# Autodesk Inventor assembly: base_assembly
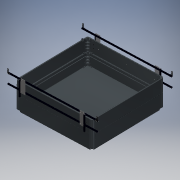
[picture p0: Inventor's stored thumbnail of the model, 180x180]
Saved by Autodesk Inventor 2018 (Build 220112000, 112)
## iProperties
Created: 2017-10-25
Part Number: base_assembly
Document SubType Name: Assembly
Designer: g
Author: g
## Documents named in this file (62)
- C:\Users\g\Desktop\AUG_inventor\base_assembly.iam
- C:\Users\g\Desktop\AUG_inventor\base_corner.ipt
- C:\Users\g\Desktop\AUG_inventor\base_wall.ipt
- C:\Users\g\Desktop\AUG_inventor\base_floor.ipt
- C:\Users\g\Desktop\AUG_inventor\makerbeam876mm.ipt
- C:\Users\g\Desktop\AUG_inventor\M3_Lock_Nut(Thin_Nut)_MIR.ipt
- C:\Users\g\Desktop\AUG_inventor\M3 X 10mm Screw_MIR.ipt
- C:\Users\g\Desktop\AUG_inventor\M3 X 10mm Screw_MIR2_MIR.ipt
- C:\Users\g\Desktop\AUG_inventor\M3_Lock_Nut(Thin_Nut)_MIR5_MIR.ipt
- C:\Users\g\Desktop\AUG_inventor\M3 X 20mm Screw_MIR_MIR_MIR1.ipt
- C:\Users\g\Desktop\AUG_inventor\M3_Lock_Nut(Thin_Nut)_MIR1_MIR_MIR1.ipt
- C:\Users\g\Desktop\AUG_inventor\makerbeam150mm_MIR_MIR_MIR_MIR1.ipt
- C:\Users\g\Desktop\AUG_inventor\M3 X 20mm Screw_MIR_MIR_MIR1_MIR.ipt
- C:\Users\g\Desktop\AUG_inventor\M3_Lock_Nut(Thin_Nut)_MIR1_MIR_MIR1_MIR.ipt
- C:\Users\g\Desktop\AUG_inventor\tieplate_small_MIR_MIR1.ipt
- C:\Users\g\Desktop\AUG_inventor\M3 X 10mm Screw_MIR2_MIR_MIR.ipt
- C:\Users\g\Desktop\AUG_inventor\M3_Lock_Nut(Thin_Nut)_MIR5_MIR_MIR.ipt
- C:\Users\g\Desktop\AUG_inventor\M3 X 20mm Screw_MIR_MIR_MIR1_MIR1.ipt
- C:\Users\g\Desktop\AUG_inventor\M3_Lock_Nut(Thin_Nut)_MIR1_MIR_MIR1_MIR1.ipt
- C:\Users\g\Desktop\AUG_inventor\makerbeam150mm_MIR_MIR_MIR_MIR1_MIR.ipt
- C:\Users\g\Desktop\AUG_inventor\M3 X 20mm Screw_MIR_MIR_MIR1_MIR_MIR.ipt
- C:\Users\g\Desktop\AUG_inventor\M3_Lock_Nut(Thin_Nut)_MIR1_MIR_MIR1_MIR_MIR.ipt
- C:\Users\g\Desktop\AUG_inventor\tieplate_small_MIR_MIR1_MIR.ipt
- C:\Users\g\Desktop\AUG_inventor\M3 X 10mm Screw_MIR2_MIR_MIR1.ipt
- C:\Users\g\Desktop\AUG_inventor\M3_Lock_Nut(Thin_Nut)_MIR5_MIR_MIR1.ipt
- C:\Users\g\Desktop\AUG_inventor\M3 X 10mm Screw_MIR2_MIR_MIR_MIR.ipt
- C:\Users\g\Desktop\AUG_inventor\M3_Lock_Nut(Thin_Nut)_MIR5_MIR_MIR_MIR.ipt
- C:\Users\g\Desktop\AUG_inventor\makerbeam876mm_MIR.ipt
- C:\Users\g\Desktop\AUG_inventor\M3_Lock_Nut(Thin_Nut)_MIR_MIR.ipt
- C:\Users\g\Desktop\AUG_inventor\M3 X 10mm Screw_MIR_MIR.ipt
- C:\Users\g\Desktop\AUG_inventor\M3 X 20mm Screw_MIR_MIR_MIR1_MIR2.ipt
- C:\Users\g\Desktop\AUG_inventor\M3_Lock_Nut(Thin_Nut)_MIR1_MIR_MIR1_MIR2.ipt
- C:\Users\g\Desktop\AUG_inventor\makerbeam150mm_MIR_MIR_MIR_MIR1_MIR1.ipt
- C:\Users\g\Desktop\AUG_inventor\M3 X 20mm Screw_MIR_MIR_MIR1_MIR_MIR1.ipt
- C:\Users\g\Desktop\AUG_inventor\M3_Lock_Nut(Thin_Nut)_MIR1_MIR_MIR1_MIR_MIR1.ipt
- C:\Users\g\Desktop\AUG_inventor\tieplate_small_MIR_MIR1_MIR1.ipt
- C:\Users\g\Desktop\AUG_inventor\M3 X 10mm Screw_MIR2_MIR_MIR2.ipt
- C:\Users\g\Desktop\AUG_inventor\M3_Lock_Nut(Thin_Nut)_MIR5_MIR_MIR2.ipt
- C:\Users\g\Desktop\AUG_inventor\M3 X 10mm Screw_MIR2_MIR_MIR_MIR1.ipt
- C:\Users\g\Desktop\AUG_inventor\M3_Lock_Nut(Thin_Nut)_MIR5_MIR_MIR_MIR1.ipt
- C:\Users\g\Desktop\AUG_inventor\M3 X 20mm Screw_MIR_MIR_MIR1_MIR1_MIR.ipt
- C:\Users\g\Desktop\AUG_inventor\M3_Lock_Nut(Thin_Nut)_MIR1_MIR_MIR1_MIR1_MIR.ipt
- C:\Users\g\Desktop\AUG_inventor\makerbeam150mm_MIR_MIR_MIR_MIR1_MIR_MIR.ipt
- C:\Users\g\Desktop\AUG_inventor\M3 X 20mm Screw_MIR_MIR_MIR1_MIR_MIR_MIR.ipt
- C:\Users\g\Desktop\AUG_inventor\M3_Lock_Nut(Thin_Nut)_MIR1_MIR_MIR1_MIR_MIR_MIR.ipt
- C:\Users\g\Desktop\AUG_inventor\tieplate_small_MIR_MIR1_MIR_MIR.ipt
- C:\Users\g\Desktop\AUG_inventor\M3 X 10mm Screw_MIR2_MIR_MIR1_MIR.ipt
- C:\Users\g\Desktop\AUG_inventor\M3_Lock_Nut(Thin_Nut)_MIR5_MIR_MIR1_MIR.ipt
- C:\Users\g\Desktop\AUG_inventor\M3 X 10mm Screw_MIR2_MIR_MIR_MIR_MIR.ipt
- C:\Users\g\Desktop\AUG_inventor\M3_Lock_Nut(Thin_Nut)_MIR5_MIR_MIR_MIR_MIR.ipt
- C:\Users\g\Desktop\AUG_inventor\makerbeam_L-bracket.ipt
- C:\Users\g\Desktop\AUG_inventor\M3_Lock_Nut(Thin_Nut).ipt
- C:\Users\g\Desktop\AUG_inventor\M3 X 10mm Screw.ipt
- C:\Users\g\Desktop\AUG_inventor\makerbeam_L-bracket_MIR2.ipt
- C:\Users\g\Desktop\AUG_inventor\M3_Lock_Nut(Thin_Nut)_MIR6.ipt
- C:\Users\g\Desktop\AUG_inventor\M3 X 10mm Screw_MIR3.ipt
- C:\Users\g\Desktop\AUG_inventor\makerbeam_L-bracket_MIR3.ipt
- C:\Users\g\Desktop\AUG_inventor\M3_Lock_Nut(Thin_Nut)_MIR7.ipt
- C:\Users\g\Desktop\AUG_inventor\M3 X 10mm Screw_MIR4.ipt
- C:\Users\g\Desktop\AUG_inventor\makerbeam_L-bracket_MIR2_MIR.ipt
- C:\Users\g\Desktop\AUG_inventor\M3_Lock_Nut(Thin_Nut)_MIR6_MIR.ipt
- C:\Users\g\Desktop\AUG_inventor\M3 X 10mm Screw_MIR3_MIR.ipt
## Components (117 placed, 61 different names)
1. base_wall:2 — Mate:1, Mate:2, Mate:9, Mate:10, Mate:15, Mate:16, Mate:23, Mate:61, Mate:62, Mate:67, Mate:68, Mate:69, Mate:114, Mate:170
2. base_wall:3 — Mate:11, Mate:12, Mate:13, Mate:14, Mate:22, Mate:57, Mate:58, Mate:63, Mate:64, Mate:70, Mate:113, Mate:123, Mate:124, Flush:2, Mate:133, Mate:145, Mate:149, Mate:164, Mate:168
3. base_wall:4 — Mate:3, Mate:4, Mate:5, Mate:6, Mate:17, Mate:18, Mate:19, Mate:24, Mate:25, Mate:60, Mate:65, Mate:66, Mate:134, Mate:135
4. base_corner:4 — Mate:1, Mate:2, Mate:3, Mate:4, Mate:16, Mate:17, Mate:23, Mate:60, Mate:61, Mate:66, Mate:67
5. base_corner:5 — Mate:13, Mate:14, Mate:57, Mate:58, Mate:64
6. base_corner:6 — Mate:5, Mate:6, Mate:7, Mate:8, Mate:18, Mate:19, Mate:20, Mate:21, Mate:24, Mate:25, Mate:26, Mate:27, Mate:28, Mate:59, Mate:65
7. base_corner:7 — Mate:9, Mate:10, Mate:11, Mate:12, Mate:15, Mate:22, Mate:62, Mate:63, Mate:68, Mate:69, Mate:70, Flush:1
8. base_wall:5 — Mate:7, Mate:8, Mate:20, Mate:21, Mate:26, Mate:27, Mate:28, Mate:59, Mate:169
9. base_wall:6 — Mate:114, Mate:116, Mate:121
10. base_wall:7 — Mate:113, Mate:118
11. base_wall:8 — Mate:122
12. base_corner:8
13. base_corner:9
14. base_corner:10
15. base_corner:11
16. base_wall:9 — Mate:117, Mate:171
17. base_floor:1 — Mate:121, Mate:122
18. makerbeam876mm:1 — Mate:124, Flush:1, Flush:2, Rigid:1, Flush:27, Mate:165, Mate:166, Mate:167, Slider:21, Flush:32, Symmetry:2
19. makerbeam876mm:4 — Rigid:1, Flush:27, Flush:28, Mate:162, Flush:29, Slider:22, Slider:23, Flush:33, Mate:173, Symmetry:2
20. M3_Lock_Nut(Thin_Nut)_MIR:1 — Slider:21, Flush:32, Cylindrical:20
21. M3_Lock_Nut(Thin_Nut)_MIR:2 — Rotational:3
22. M3_Lock_Nut(Thin_Nut)_MIR:3 — Rigid:4
23. M3 X 10mm Screw_MIR:1 — Rotational:3, Mate:145
24. M3 X 10mm Screw_MIR:2 — Cylindrical:20, Mate:168
25. M3 X 10mm Screw_MIR:3 — Rigid:4, Mate:149
26. M3 X 20mm Screw_MIR_MIR_MIR1:1 — Cylindrical:18, Mate:164
27. M3_Lock_Nut(Thin_Nut)_MIR1_MIR_MIR1:1 — Slider:20, Flush:31, Cylindrical:18
28. makerbeam150mm_MIR_MIR_MIR_MIR1:1 — Flush:28, Mate:162, Flush:29, Slider:20, Flush:31, Mate:172, Mate:174
29. M3 X 20mm Screw_MIR_MIR_MIR1_MIR:1 — Cylindrical:19
30. M3_Lock_Nut(Thin_Nut)_MIR1_MIR_MIR1_MIR:1 — Cylindrical:19
31. tieplate_small_MIR_MIR1:1 — Flush:33, Mate:173, Mate:174, Mate:175, Mate:176, Mate:177
32. M3 X 10mm Screw_MIR2_MIR:1 — Cylindrical:22, Mate:176
33. M3_Lock_Nut(Thin_Nut)_MIR5_MIR:1 — Slider:23, Cylindrical:22, Mate:175
34. M3_Lock_Nut(Thin_Nut)_MIR5_MIR:2 — Slider:22, Mate:172, Cylindrical:21
35. M3 X 10mm Screw_MIR2_MIR:2 — Cylindrical:21, Mate:177
36. M3 X 10mm Screw_MIR2_MIR_MIR:1 — Cylindrical:23
37. M3_Lock_Nut(Thin_Nut)_MIR5_MIR_MIR:1 — Cylindrical:23
38. M3_Lock_Nut(Thin_Nut)_MIR5_MIR_MIR:2 — Cylindrical:24
39. M3 X 10mm Screw_MIR2_MIR_MIR:2 — Cylindrical:24
40. M3 X 20mm Screw_MIR_MIR_MIR1_MIR1:1 — Cylindrical:25
41. M3_Lock_Nut(Thin_Nut)_MIR1_MIR_MIR1_MIR1:1 — Flush:34, Cylindrical:25, Slider:24
42. makerbeam150mm_MIR_MIR_MIR_MIR1_MIR:1 — Flush:34, Mate:178, Mate:181, Slider:24
43. M3 X 20mm Screw_MIR_MIR_MIR1_MIR_MIR:1 — Cylindrical:26
44. M3_Lock_Nut(Thin_Nut)_MIR1_MIR_MIR1_MIR_MIR:1 — Cylindrical:26
45. tieplate_small_MIR_MIR1_MIR:1 — Mate:178, Mate:179, Mate:180, Mate:182
46. M3 X 10mm Screw_MIR2_MIR_MIR1:1 — Mate:179, Cylindrical:27
47. M3_Lock_Nut(Thin_Nut)_MIR5_MIR_MIR1:1 — Mate:180, Cylindrical:27
48. M3_Lock_Nut(Thin_Nut)_MIR5_MIR_MIR1:2 — Mate:181, Cylindrical:28
49. M3 X 10mm Screw_MIR2_MIR_MIR1:2 — Mate:182, Cylindrical:28
50. M3 X 10mm Screw_MIR2_MIR_MIR_MIR:1 — Cylindrical:29
51. M3_Lock_Nut(Thin_Nut)_MIR5_MIR_MIR_MIR:1 — Cylindrical:29
52. M3_Lock_Nut(Thin_Nut)_MIR5_MIR_MIR_MIR:2 — Cylindrical:30
53. M3 X 10mm Screw_MIR2_MIR_MIR_MIR:2 — Cylindrical:30
54. makerbeam876mm_MIR:1 — Flush:35, Flush:36, Mate:184, Mate:185, Mate:186, Symmetry:3, Rigid:5, Slider:25
55. makerbeam876mm_MIR:2 — Flush:35, Flush:38, Mate:183, Flush:39, Mate:188, Flush:40, Symmetry:3, Rigid:5, Slider:27, Slider:28, Slider:30, Flush:42, Slider:31, Mate:198, Flush:43, Flush:44
56. M3_Lock_Nut(Thin_Nut)_MIR_MIR:1 — Flush:36, Slider:25, Cylindrical:31
57. M3_Lock_Nut(Thin_Nut)_MIR_MIR:2 — Rotational:4
58. M3_Lock_Nut(Thin_Nut)_MIR_MIR:3 — Rigid:6
59. M3 X 10mm Screw_MIR_MIR:1 — Rotational:4
60. M3 X 10mm Screw_MIR_MIR:2 — Cylindrical:31
61. M3 X 10mm Screw_MIR_MIR:3 — Rigid:6
62. M3 X 20mm Screw_MIR_MIR_MIR1_MIR2:1 — Cylindrical:32
63. M3_Lock_Nut(Thin_Nut)_MIR1_MIR_MIR1_MIR2:1 — Flush:37, Cylindrical:32, Slider:26
64. makerbeam150mm_MIR_MIR_MIR_MIR1_MIR1:1 — Flush:37, Flush:38, Mate:183, Flush:39, Mate:187, Mate:191, Slider:26
65. M3 X 20mm Screw_MIR_MIR_MIR1_MIR_MIR1:1 — Cylindrical:33
66. M3_Lock_Nut(Thin_Nut)_MIR1_MIR_MIR1_MIR_MIR1:1 — Cylindrical:33
67. tieplate_small_MIR_MIR1_MIR1:1 — Mate:187, Mate:188, Flush:40, Mate:189, Mate:190, Mate:192
68. M3 X 10mm Screw_MIR2_MIR_MIR2:1 — Mate:189, Cylindrical:34
69. M3_Lock_Nut(Thin_Nut)_MIR5_MIR_MIR2:1 — Mate:190, Cylindrical:34, Slider:27
70. M3_Lock_Nut(Thin_Nut)_MIR5_MIR_MIR2:2 — Mate:191, Slider:28, Cylindrical:35
71. M3 X 10mm Screw_MIR2_MIR_MIR2:2 — Mate:192, Cylindrical:35
72. M3 X 10mm Screw_MIR2_MIR_MIR_MIR1:1 — Cylindrical:36
73. M3_Lock_Nut(Thin_Nut)_MIR5_MIR_MIR_MIR1:1 — Cylindrical:36
74. M3_Lock_Nut(Thin_Nut)_MIR5_MIR_MIR_MIR1:2 — Cylindrical:37
75. M3 X 10mm Screw_MIR2_MIR_MIR_MIR1:2 — Cylindrical:37
76. M3 X 20mm Screw_MIR_MIR_MIR1_MIR1_MIR:1 — Cylindrical:38
77. M3_Lock_Nut(Thin_Nut)_MIR1_MIR_MIR1_MIR1_MIR:1 — Flush:41, Cylindrical:38, Slider:29
78. makerbeam150mm_MIR_MIR_MIR_MIR1_MIR_MIR:1 — Flush:41, Mate:193, Mate:196, Slider:29
79. M3 X 20mm Screw_MIR_MIR_MIR1_MIR_MIR_MIR:1 — Cylindrical:39
80. M3_Lock_Nut(Thin_Nut)_MIR1_MIR_MIR1_MIR_MIR_MIR:1 — Cylindrical:39
81. tieplate_small_MIR_MIR1_MIR_MIR:1 — Mate:193, Mate:194, Mate:195, Mate:197
82. M3 X 10mm Screw_MIR2_MIR_MIR1_MIR:1 — Mate:194, Cylindrical:40
83. M3_Lock_Nut(Thin_Nut)_MIR5_MIR_MIR1_MIR:1 — Mate:195, Cylindrical:40
84. M3_Lock_Nut(Thin_Nut)_MIR5_MIR_MIR1_MIR:2 — Mate:196, Cylindrical:41
85. M3 X 10mm Screw_MIR2_MIR_MIR1_MIR:2 — Mate:197, Cylindrical:41
86. M3 X 10mm Screw_MIR2_MIR_MIR_MIR_MIR:1 — Cylindrical:42
87. M3_Lock_Nut(Thin_Nut)_MIR5_MIR_MIR_MIR_MIR:1 — Cylindrical:42
88. M3_Lock_Nut(Thin_Nut)_MIR5_MIR_MIR_MIR_MIR:2 — Cylindrical:43
89. M3 X 10mm Screw_MIR2_MIR_MIR_MIR_MIR:2 — Cylindrical:43
90. makerbeam_L-bracket:1 — Mate:198, Flush:43, Flush:44, Mate:199, Mate:200, Mate:201, Mate:202, Cylindrical:46, Mate:203
91. M3_Lock_Nut(Thin_Nut):1 — Slider:30, Flush:42, Cylindrical:45
92. M3_Lock_Nut(Thin_Nut):2 — Slider:31, Mate:199, Cylindrical:44
93. M3 X 10mm Screw:1 — Cylindrical:44, Mate:200
94. M3 X 10mm Screw:2 — Cylindrical:45, Mate:201
95. M3_Lock_Nut(Thin_Nut):3 — Mate:202
96. M3 X 10mm Screw:3 — Cylindrical:46, Mate:203
97. makerbeam_L-bracket_MIR2:1 — Mate:204, Mate:205, Mate:206, Mate:207, Mate:208, Cylindrical:49
98. M3_Lock_Nut(Thin_Nut)_MIR6:1 — Cylindrical:48
99. M3_Lock_Nut(Thin_Nut)_MIR6:2 — Mate:204, Cylindrical:47
100. M3 X 10mm Screw_MIR3:1 — Mate:205, Cylindrical:47
101. M3 X 10mm Screw_MIR3:2 — Mate:206, Cylindrical:48
102. M3_Lock_Nut(Thin_Nut)_MIR6:3 — Mate:207
103. M3 X 10mm Screw_MIR3:3 — Mate:208, Cylindrical:49
104. makerbeam_L-bracket_MIR3:1 — Mate:209, Mate:210, Mate:211, Mate:212, Mate:213, Cylindrical:52
105. M3_Lock_Nut(Thin_Nut)_MIR7:1 — Cylindrical:51
106. M3_Lock_Nut(Thin_Nut)_MIR7:2 — Mate:209, Cylindrical:50
107. M3 X 10mm Screw_MIR4:1 — Mate:210, Cylindrical:50
108. M3 X 10mm Screw_MIR4:2 — Mate:211, Cylindrical:51
109. M3_Lock_Nut(Thin_Nut)_MIR7:3 — Mate:212
110. M3 X 10mm Screw_MIR4:3 — Mate:213, Cylindrical:52
111. makerbeam_L-bracket_MIR2_MIR:1 — Mate:214, Mate:215, Mate:216, Mate:217, Mate:218, Cylindrical:55
112. M3_Lock_Nut(Thin_Nut)_MIR6_MIR:1 — Cylindrical:54
113. M3_Lock_Nut(Thin_Nut)_MIR6_MIR:2 — Mate:214, Cylindrical:53
114. M3 X 10mm Screw_MIR3_MIR:1 — Mate:215, Cylindrical:53
115. M3 X 10mm Screw_MIR3_MIR:2 — Mate:216, Cylindrical:54
116. M3_Lock_Nut(Thin_Nut)_MIR6_MIR:3 — Mate:217
117. M3 X 10mm Screw_MIR3_MIR:3 — Mate:218, Cylindrical:55
## Relationships (233: Mate 156, CylindricalJoint 38, Flush 19, TranslationJoint 12, WeldJoint 4, RevoluteJoint 2, Symmetry 2)
- Mate:1: base_wall:2 ↔ base_corner:4
- Mate:2: base_wall:2 ↔ base_corner:4
- Mate:3: base_wall:4 ↔ base_corner:4
- Mate:4: base_wall:4 ↔ base_corner:4
- Mate:5: base_wall:4 ↔ base_corner:6
- Mate:6: base_wall:4 ↔ base_corner:6
- Mate:7: base_corner:6 ↔ base_wall:5
- Mate:8: base_corner:6 ↔ base_wall:5
- Mate:9: base_wall:2 ↔ base_corner:7
- Mate:10: base_wall:2 ↔ base_corner:7
- Mate:11: base_wall:3 ↔ base_corner:7
- Mate:12: base_wall:3 ↔ base_corner:7
- Mate:13: base_wall:3 ↔ base_corner:5
- Mate:14: base_wall:3 ↔ base_corner:5
- Mate:15: base_wall:2 ↔ base_corner:7
- Mate:16: base_wall:2 ↔ base_corner:4
- Mate:17: base_wall:4 ↔ base_corner:4
- Mate:18: base_wall:4 ↔ base_corner:6
- Mate:19: base_wall:4 ↔ base_corner:6
- Mate:20: base_corner:6 ↔ base_wall:5
- Mate:21: base_corner:6 ↔ base_wall:5
- Mate:22: base_wall:3 ↔ base_corner:7
- Mate:23: base_wall:2 ↔ base_corner:4
- Mate:24: base_wall:4 ↔ base_corner:6
- Mate:25: base_wall:4 ↔ base_corner:6
- Mate:26: base_corner:6 ↔ base_wall:5
- Mate:27: base_corner:6 ↔ base_wall:5
- Mate:28: base_corner:6 ↔ base_wall:5
- Mate:57: base_wall:3 ↔ base_corner:5
- Mate:58: base_wall:3 ↔ base_corner:5
- Mate:59: base_corner:6 ↔ base_wall:5
- Mate:60: base_wall:4 ↔ base_corner:4
- Mate:61: base_wall:2 ↔ base_corner:4
- Mate:62: base_wall:2 ↔ base_corner:7
- Mate:63: base_wall:3 ↔ base_corner:7
- Mate:64: base_wall:3 ↔ base_corner:5
- Mate:65: base_wall:4 ↔ base_corner:6
- Mate:66: base_wall:4 ↔ base_corner:4
- Mate:67: base_wall:2 ↔ base_corner:4
- Mate:68: base_wall:2 ↔ base_corner:7
- Mate:69: base_wall:2 ↔ base_corner:7
- Mate:70: base_wall:3 ↔ base_corner:7
- [Mate]: base_wall:6 ↔ base_corner:8
- [Mate]: base_wall:6 ↔ base_corner:8
- [Mate]: base_wall:8 ↔ base_corner:8
- [Mate]: base_wall:8 ↔ base_corner:8
- [Mate]: base_wall:8 ↔ base_corner:10
- [Mate]: base_wall:8 ↔ base_corner:10
- [Mate]: base_corner:10 ↔ base_wall:9
- [Mate]: base_corner:10 ↔ base_wall:9
- [Mate]: base_wall:6 ↔ base_corner:11
- [Mate]: base_wall:6 ↔ base_corner:11
- [Mate]: base_wall:7 ↔ base_corner:11
- [Mate]: base_wall:7 ↔ base_corner:11
- [Mate]: base_wall:7 ↔ base_corner:9
- [Mate]: base_wall:7 ↔ base_corner:9
- [Mate]: base_wall:6 ↔ base_corner:11
- [Mate]: base_wall:6 ↔ base_corner:8
- [Mate]: base_wall:8 ↔ base_corner:8
- [Mate]: base_wall:8 ↔ base_corner:10
- [Mate]: base_wall:8 ↔ base_corner:10
- [Mate]: base_corner:10 ↔ base_wall:9
- [Mate]: base_corner:10 ↔ base_wall:9
- [Mate]: base_wall:7 ↔ base_corner:11
- [Mate]: base_wall:6 ↔ base_corner:8
- [Mate]: base_wall:8 ↔ base_corner:10
- [Mate]: base_wall:8 ↔ base_corner:10
- [Mate]: base_corner:10 ↔ base_wall:9
- [Mate]: base_corner:10 ↔ base_wall:9
- [Mate]: base_corner:10 ↔ base_wall:9
- [Mate]: base_wall:7 ↔ base_corner:9
- [Mate]: base_wall:7 ↔ base_corner:9
- [Mate]: base_corner:10 ↔ base_wall:9
- [Mate]: base_wall:8 ↔ base_corner:8
- [Mate]: base_wall:6 ↔ base_corner:8
- [Mate]: base_wall:6 ↔ base_corner:11
- [Mate]: base_wall:7 ↔ base_corner:11
- [Mate]: base_wall:7 ↔ base_corner:9
- [Mate]: base_wall:8 ↔ base_corner:10
- [Mate]: base_wall:8 ↔ base_corner:8
- [Mate]: base_wall:6 ↔ base_corner:8
- [Mate]: base_wall:6 ↔ base_corner:11
- [Mate]: base_wall:6 ↔ base_corner:11
- [Mate]: base_wall:7 ↔ base_corner:11
- Mate:113: base_wall:3 ↔ base_wall:7
- Mate:114: base_wall:2 ↔ base_wall:6
- Mate:116: base_wall:6
- Mate:117: base_wall:9
- Mate:118: base_wall:7
- Mate:119
- Mate:120
- Mate:121: base_wall:6 ↔ base_floor:1
- Mate:122: base_wall:8 ↔ base_floor:1
- Mate:123: base_wall:3
- Mate:124 (5 mm): base_wall:3 ↔ makerbeam876mm:1
- Flush:1 (-68 mm): base_corner:7 ↔ makerbeam876mm:1
- Flush:2 (57.5 mm): base_wall:3 ↔ makerbeam876mm:1
- Rigid:1 [WeldJoint] (85 mm): makerbeam876mm:1 ↔ makerbeam876mm:4
- Rotational:3 [RevoluteJoint] (2.55 mm): M3_Lock_Nut(Thin_Nut)_MIR:2 ↔ M3 X 10mm Screw_MIR:1
- Rigid:4 [WeldJoint] (-2.54 mm): M3_Lock_Nut(Thin_Nut)_MIR:3 ↔ M3 X 10mm Screw_MIR:3
- Mate:133: base_wall:3
- Mate:134: base_wall:4
- Mate:135: base_wall:4
- Mate:145: base_wall:3 ↔ M3 X 10mm Screw_MIR:1
- Mate:149: base_wall:3 ↔ M3 X 10mm Screw_MIR:3
- Flush:27: makerbeam876mm:1 ↔ makerbeam876mm:4
- Flush:28: makerbeam876mm:4 ↔ makerbeam150mm_MIR_MIR_MIR_MIR1:1
- Mate:162: makerbeam876mm:4 ↔ makerbeam150mm_MIR_MIR_MIR_MIR1:1
- Flush:29 (120 mm): makerbeam876mm:4 ↔ makerbeam150mm_MIR_MIR_MIR_MIR1:1
- Slider:20 [TranslationJoint] (0.25 mm): M3_Lock_Nut(Thin_Nut)_MIR1_MIR_MIR1:1 ↔ makerbeam150mm_MIR_MIR_MIR_MIR1:1
- Flush:31 (80 mm): M3_Lock_Nut(Thin_Nut)_MIR1_MIR_MIR1:1 ↔ makerbeam150mm_MIR_MIR_MIR_MIR1:1
- Cylindrical:18: M3 X 20mm Screw_MIR_MIR_MIR1:1 ↔ M3_Lock_Nut(Thin_Nut)_MIR1_MIR_MIR1:1
- Mate:164: base_wall:3 ↔ M3 X 20mm Screw_MIR_MIR_MIR1:1
- Mate:165: makerbeam876mm:1
- Mate:166: makerbeam876mm:1
- Mate:167: makerbeam876mm:1
- Cylindrical:19: M3 X 20mm Screw_MIR_MIR_MIR1_MIR:1 ↔ M3_Lock_Nut(Thin_Nut)_MIR1_MIR_MIR1_MIR:1
- Slider:21 [TranslationJoint]: makerbeam876mm:1 ↔ M3_Lock_Nut(Thin_Nut)_MIR:1
- Flush:32 (168 mm): makerbeam876mm:1 ↔ M3_Lock_Nut(Thin_Nut)_MIR:1
- Cylindrical:20: M3_Lock_Nut(Thin_Nut)_MIR:1 ↔ M3 X 10mm Screw_MIR:2
- Mate:168: base_wall:3 ↔ M3 X 10mm Screw_MIR:2
- Mate:169: base_wall:5
- Mate:170: base_wall:2
- Mate:171: base_wall:9
- Slider:22 [TranslationJoint]: makerbeam876mm:4 ↔ M3_Lock_Nut(Thin_Nut)_MIR5_MIR:2
- Mate:172 (5 mm): makerbeam150mm_MIR_MIR_MIR_MIR1:1 ↔ M3_Lock_Nut(Thin_Nut)_MIR5_MIR:2
- Slider:23 [TranslationJoint]: makerbeam876mm:4 ↔ M3_Lock_Nut(Thin_Nut)_MIR5_MIR:1
- Flush:33 (-10 mm): makerbeam876mm:4 ↔ tieplate_small_MIR_MIR1:1
- Mate:173: makerbeam876mm:4 ↔ tieplate_small_MIR_MIR1:1
- Cylindrical:21: M3_Lock_Nut(Thin_Nut)_MIR5_MIR:2 ↔ M3 X 10mm Screw_MIR2_MIR:2
- Cylindrical:22: M3 X 10mm Screw_MIR2_MIR:1 ↔ M3_Lock_Nut(Thin_Nut)_MIR5_MIR:1
- Mate:174: makerbeam150mm_MIR_MIR_MIR_MIR1:1 ↔ tieplate_small_MIR_MIR1:1
- Mate:175 (-10.25 mm): tieplate_small_MIR_MIR1:1 ↔ M3_Lock_Nut(Thin_Nut)_MIR5_MIR:1
- Symmetry:2: makerbeam876mm:1 ↔ makerbeam876mm:4
- Mate:176: tieplate_small_MIR_MIR1:1 ↔ M3 X 10mm Screw_MIR2_MIR:1
- Mate:177: tieplate_small_MIR_MIR1:1 ↔ M3 X 10mm Screw_MIR2_MIR:2
- Cylindrical:23: M3 X 10mm Screw_MIR2_MIR_MIR:1 ↔ M3_Lock_Nut(Thin_Nut)_MIR5_MIR_MIR:1
- Cylindrical:24: M3_Lock_Nut(Thin_Nut)_MIR5_MIR_MIR:2 ↔ M3 X 10mm Screw_MIR2_MIR_MIR:2
- Flush:34 (80 mm): M3_Lock_Nut(Thin_Nut)_MIR1_MIR_MIR1_MIR1:1 ↔ makerbeam150mm_MIR_MIR_MIR_MIR1_MIR:1
- Mate:178: makerbeam150mm_MIR_MIR_MIR_MIR1_MIR:1 ↔ tieplate_small_MIR_MIR1_MIR:1
- Mate:179: tieplate_small_MIR_MIR1_MIR:1 ↔ M3 X 10mm Screw_MIR2_MIR_MIR1:1
- Mate:180 (-10.25 mm): tieplate_small_MIR_MIR1_MIR:1 ↔ M3_Lock_Nut(Thin_Nut)_MIR5_MIR_MIR1:1
- Mate:181 (5 mm): makerbeam150mm_MIR_MIR_MIR_MIR1_MIR:1 ↔ M3_Lock_Nut(Thin_Nut)_MIR5_MIR_MIR1:2
- Mate:182: tieplate_small_MIR_MIR1_MIR:1 ↔ M3 X 10mm Screw_MIR2_MIR_MIR1:2
- Cylindrical:25: M3 X 20mm Screw_MIR_MIR_MIR1_MIR1:1 ↔ M3_Lock_Nut(Thin_Nut)_MIR1_MIR_MIR1_MIR1:1
- Slider:24 [TranslationJoint] (0.25 mm): M3_Lock_Nut(Thin_Nut)_MIR1_MIR_MIR1_MIR1:1 ↔ makerbeam150mm_MIR_MIR_MIR_MIR1_MIR:1
- Cylindrical:26: M3 X 20mm Screw_MIR_MIR_MIR1_MIR_MIR:1 ↔ M3_Lock_Nut(Thin_Nut)_MIR1_MIR_MIR1_MIR_MIR:1
- Cylindrical:27: M3 X 10mm Screw_MIR2_MIR_MIR1:1 ↔ M3_Lock_Nut(Thin_Nut)_MIR5_MIR_MIR1:1
- Cylindrical:28: M3_Lock_Nut(Thin_Nut)_MIR5_MIR_MIR1:2 ↔ M3 X 10mm Screw_MIR2_MIR_MIR1:2
- Cylindrical:29: M3 X 10mm Screw_MIR2_MIR_MIR_MIR:1 ↔ M3_Lock_Nut(Thin_Nut)_MIR5_MIR_MIR_MIR:1
- Cylindrical:30: M3_Lock_Nut(Thin_Nut)_MIR5_MIR_MIR_MIR:2 ↔ M3 X 10mm Screw_MIR2_MIR_MIR_MIR:2
- Flush:35: makerbeam876mm_MIR:1 ↔ makerbeam876mm_MIR:2
- Flush:36 (168 mm): makerbeam876mm_MIR:1 ↔ M3_Lock_Nut(Thin_Nut)_MIR_MIR:1
- Flush:37 (80 mm): M3_Lock_Nut(Thin_Nut)_MIR1_MIR_MIR1_MIR2:1 ↔ makerbeam150mm_MIR_MIR_MIR_MIR1_MIR1:1
- Flush:38 (120 mm): makerbeam876mm_MIR:2 ↔ makerbeam150mm_MIR_MIR_MIR_MIR1_MIR1:1
- Mate:183: makerbeam876mm_MIR:2 ↔ makerbeam150mm_MIR_MIR_MIR_MIR1_MIR1:1
- Flush:39: makerbeam876mm_MIR:2 ↔ makerbeam150mm_MIR_MIR_MIR_MIR1_MIR1:1
- Mate:184: makerbeam876mm_MIR:1
- Mate:185: makerbeam876mm_MIR:1
- Mate:186: makerbeam876mm_MIR:1
- Mate:187: makerbeam150mm_MIR_MIR_MIR_MIR1_MIR1:1 ↔ tieplate_small_MIR_MIR1_MIR1:1
- Mate:188: makerbeam876mm_MIR:2 ↔ tieplate_small_MIR_MIR1_MIR1:1
- Flush:40 (-10 mm): makerbeam876mm_MIR:2 ↔ tieplate_small_MIR_MIR1_MIR1:1
- Mate:189: tieplate_small_MIR_MIR1_MIR1:1 ↔ M3 X 10mm Screw_MIR2_MIR_MIR2:1
- Mate:190 (-10.25 mm): tieplate_small_MIR_MIR1_MIR1:1 ↔ M3_Lock_Nut(Thin_Nut)_MIR5_MIR_MIR2:1
- Mate:191 (5 mm): makerbeam150mm_MIR_MIR_MIR_MIR1_MIR1:1 ↔ M3_Lock_Nut(Thin_Nut)_MIR5_MIR_MIR2:2
- Mate:192: tieplate_small_MIR_MIR1_MIR1:1 ↔ M3 X 10mm Screw_MIR2_MIR_MIR2:2
- Symmetry:3: makerbeam876mm_MIR:1 ↔ makerbeam876mm_MIR:2
- Flush:41 (80 mm): M3_Lock_Nut(Thin_Nut)_MIR1_MIR_MIR1_MIR1_MIR:1 ↔ makerbeam150mm_MIR_MIR_MIR_MIR1_MIR_MIR:1
- Mate:193: makerbeam150mm_MIR_MIR_MIR_MIR1_MIR_MIR:1 ↔ tieplate_small_MIR_MIR1_MIR_MIR:1
- Mate:194: tieplate_small_MIR_MIR1_MIR_MIR:1 ↔ M3 X 10mm Screw_MIR2_MIR_MIR1_MIR:1
- Mate:195 (-10.25 mm): tieplate_small_MIR_MIR1_MIR_MIR:1 ↔ M3_Lock_Nut(Thin_Nut)_MIR5_MIR_MIR1_MIR:1
- Mate:196 (5 mm): makerbeam150mm_MIR_MIR_MIR_MIR1_MIR_MIR:1 ↔ M3_Lock_Nut(Thin_Nut)_MIR5_MIR_MIR1_MIR:2
- Mate:197: tieplate_small_MIR_MIR1_MIR_MIR:1 ↔ M3 X 10mm Screw_MIR2_MIR_MIR1_MIR:2
- Rigid:5 [WeldJoint] (85 mm): makerbeam876mm_MIR:1 ↔ makerbeam876mm_MIR:2
- Slider:25 [TranslationJoint]: makerbeam876mm_MIR:1 ↔ M3_Lock_Nut(Thin_Nut)_MIR_MIR:1
- Rotational:4 [RevoluteJoint] (-2.55 mm): M3_Lock_Nut(Thin_Nut)_MIR_MIR:2 ↔ M3 X 10mm Screw_MIR_MIR:1
- Cylindrical:31: M3_Lock_Nut(Thin_Nut)_MIR_MIR:1 ↔ M3 X 10mm Screw_MIR_MIR:2
- Rigid:6 [WeldJoint] (-2.54 mm): M3_Lock_Nut(Thin_Nut)_MIR_MIR:3 ↔ M3 X 10mm Screw_MIR_MIR:3
- Cylindrical:32: M3 X 20mm Screw_MIR_MIR_MIR1_MIR2:1 ↔ M3_Lock_Nut(Thin_Nut)_MIR1_MIR_MIR1_MIR2:1
- Slider:26 [TranslationJoint] (0.25 mm): M3_Lock_Nut(Thin_Nut)_MIR1_MIR_MIR1_MIR2:1 ↔ makerbeam150mm_MIR_MIR_MIR_MIR1_MIR1:1
- Cylindrical:33: M3 X 20mm Screw_MIR_MIR_MIR1_MIR_MIR1:1 ↔ M3_Lock_Nut(Thin_Nut)_MIR1_MIR_MIR1_MIR_MIR1:1
- Cylindrical:34: M3 X 10mm Screw_MIR2_MIR_MIR2:1 ↔ M3_Lock_Nut(Thin_Nut)_MIR5_MIR_MIR2:1
- Slider:27 [TranslationJoint]: makerbeam876mm_MIR:2 ↔ M3_Lock_Nut(Thin_Nut)_MIR5_MIR_MIR2:1
- Slider:28 [TranslationJoint]: makerbeam876mm_MIR:2 ↔ M3_Lock_Nut(Thin_Nut)_MIR5_MIR_MIR2:2
- Cylindrical:35: M3_Lock_Nut(Thin_Nut)_MIR5_MIR_MIR2:2 ↔ M3 X 10mm Screw_MIR2_MIR_MIR2:2
- Cylindrical:36: M3 X 10mm Screw_MIR2_MIR_MIR_MIR1:1 ↔ M3_Lock_Nut(Thin_Nut)_MIR5_MIR_MIR_MIR1:1
- Cylindrical:37: M3_Lock_Nut(Thin_Nut)_MIR5_MIR_MIR_MIR1:2 ↔ M3 X 10mm Screw_MIR2_MIR_MIR_MIR1:2
- Cylindrical:38: M3 X 20mm Screw_MIR_MIR_MIR1_MIR1_MIR:1 ↔ M3_Lock_Nut(Thin_Nut)_MIR1_MIR_MIR1_MIR1_MIR:1
- Slider:29 [TranslationJoint] (0.25 mm): M3_Lock_Nut(Thin_Nut)_MIR1_MIR_MIR1_MIR1_MIR:1 ↔ makerbeam150mm_MIR_MIR_MIR_MIR1_MIR_MIR:1
- Cylindrical:39: M3 X 20mm Screw_MIR_MIR_MIR1_MIR_MIR_MIR:1 ↔ M3_Lock_Nut(Thin_Nut)_MIR1_MIR_MIR1_MIR_MIR_MIR:1
- Cylindrical:40: M3 X 10mm Screw_MIR2_MIR_MIR1_MIR:1 ↔ M3_Lock_Nut(Thin_Nut)_MIR5_MIR_MIR1_MIR:1
- Cylindrical:41: M3_Lock_Nut(Thin_Nut)_MIR5_MIR_MIR1_MIR:2 ↔ M3 X 10mm Screw_MIR2_MIR_MIR1_MIR:2
- Cylindrical:42: M3 X 10mm Screw_MIR2_MIR_MIR_MIR_MIR:1 ↔ M3_Lock_Nut(Thin_Nut)_MIR5_MIR_MIR_MIR_MIR:1
- Cylindrical:43: M3_Lock_Nut(Thin_Nut)_MIR5_MIR_MIR_MIR_MIR:2 ↔ M3 X 10mm Screw_MIR2_MIR_MIR_MIR_MIR:2
- Slider:30 [TranslationJoint]: makerbeam876mm_MIR:2 ↔ M3_Lock_Nut(Thin_Nut):1
- Flush:42 (2.25 mm): makerbeam876mm_MIR:2 ↔ M3_Lock_Nut(Thin_Nut):1
- Slider:31 [TranslationJoint]: makerbeam876mm_MIR:2 ↔ M3_Lock_Nut(Thin_Nut):2
- Mate:198: makerbeam876mm_MIR:2 ↔ makerbeam_L-bracket:1
- Flush:43: makerbeam876mm_MIR:2 ↔ makerbeam_L-bracket:1
- Flush:44: makerbeam876mm_MIR:2 ↔ makerbeam_L-bracket:1
- Mate:199 (-7.75 mm): makerbeam_L-bracket:1 ↔ M3_Lock_Nut(Thin_Nut):2
- Cylindrical:44: M3_Lock_Nut(Thin_Nut):2 ↔ M3 X 10mm Screw:1
- Cylindrical:45: M3_Lock_Nut(Thin_Nut):1 ↔ M3 X 10mm Screw:2
- Mate:200: makerbeam_L-bracket:1 ↔ M3 X 10mm Screw:1
- Mate:201: makerbeam_L-bracket:1 ↔ M3 X 10mm Screw:2
- Mate:202: makerbeam_L-bracket:1 ↔ M3_Lock_Nut(Thin_Nut):3
- Cylindrical:46: makerbeam_L-bracket:1 ↔ M3 X 10mm Screw:3
- Mate:203: makerbeam_L-bracket:1 ↔ M3 X 10mm Screw:3
- Mate:204 (-7.75 mm): makerbeam_L-bracket_MIR2:1 ↔ M3_Lock_Nut(Thin_Nut)_MIR6:2
- Mate:205: makerbeam_L-bracket_MIR2:1 ↔ M3 X 10mm Screw_MIR3:1
- Mate:206: makerbeam_L-bracket_MIR2:1 ↔ M3 X 10mm Screw_MIR3:2
- Mate:207: makerbeam_L-bracket_MIR2:1 ↔ M3_Lock_Nut(Thin_Nut)_MIR6:3
- Mate:208: makerbeam_L-bracket_MIR2:1 ↔ M3 X 10mm Screw_MIR3:3
- Cylindrical:47: M3_Lock_Nut(Thin_Nut)_MIR6:2 ↔ M3 X 10mm Screw_MIR3:1
- Cylindrical:48: M3_Lock_Nut(Thin_Nut)_MIR6:1 ↔ M3 X 10mm Screw_MIR3:2
- Cylindrical:49: makerbeam_L-bracket_MIR2:1 ↔ M3 X 10mm Screw_MIR3:3
- Mate:209 (-7.75 mm): makerbeam_L-bracket_MIR3:1 ↔ M3_Lock_Nut(Thin_Nut)_MIR7:2
- Mate:210: makerbeam_L-bracket_MIR3:1 ↔ M3 X 10mm Screw_MIR4:1
- Mate:211: makerbeam_L-bracket_MIR3:1 ↔ M3 X 10mm Screw_MIR4:2
- Mate:212: makerbeam_L-bracket_MIR3:1 ↔ M3_Lock_Nut(Thin_Nut)_MIR7:3
- Mate:213: makerbeam_L-bracket_MIR3:1 ↔ M3 X 10mm Screw_MIR4:3
- Mate:214 (-7.75 mm): makerbeam_L-bracket_MIR2_MIR:1 ↔ M3_Lock_Nut(Thin_Nut)_MIR6_MIR:2
- Mate:215: makerbeam_L-bracket_MIR2_MIR:1 ↔ M3 X 10mm Screw_MIR3_MIR:1
- Mate:216: makerbeam_L-bracket_MIR2_MIR:1 ↔ M3 X 10mm Screw_MIR3_MIR:2
- Mate:217: makerbeam_L-bracket_MIR2_MIR:1 ↔ M3_Lock_Nut(Thin_Nut)_MIR6_MIR:3
- Mate:218: makerbeam_L-bracket_MIR2_MIR:1 ↔ M3 X 10mm Screw_MIR3_MIR:3
- Cylindrical:50: M3_Lock_Nut(Thin_Nut)_MIR7:2 ↔ M3 X 10mm Screw_MIR4:1
- Cylindrical:51: M3_Lock_Nut(Thin_Nut)_MIR7:1 ↔ M3 X 10mm Screw_MIR4:2
- Cylindrical:52: makerbeam_L-bracket_MIR3:1 ↔ M3 X 10mm Screw_MIR4:3
- Cylindrical:53: M3_Lock_Nut(Thin_Nut)_MIR6_MIR:2 ↔ M3 X 10mm Screw_MIR3_MIR:1
- Cylindrical:54: M3_Lock_Nut(Thin_Nut)_MIR6_MIR:1 ↔ M3 X 10mm Screw_MIR3_MIR:2
- Cylindrical:55: makerbeam_L-bracket_MIR2_MIR:1 ↔ M3 X 10mm Screw_MIR3_MIR:3
## Named parameters: d70_d63 = 0 mm, d71_d64 = 0 mm, d72_d65 = 0 mm, d73_d66 = 0 mm, d74_d67 = 0 mm, d75_d68 = 0 mm, d76_d69 = 0 mm, d77_d56 = 0 mm, d78_d57 = 0 mm, d79_d58 = 0 mm, d80_d59 = 0 mm, d81_d60 = 0 mm, d82_d61 = 0 mm, d83_d62 = 0 mm, d84_d21 = 0 mm, d85_d22 = 0 mm, d86_d23 = 0 mm, d87_d24 = 0 mm, d88_d25 = 0 mm, d89_d26 = 0 mm, d90_d27 = 0 mm, d91_d11 = 0 mm, d92_d12 = 0 mm, d93_d13 = 0 mm, d94_d14 = 0 mm, d95_d15 = 0 mm, d96_d16 = 0 mm, d97_d17 = 0 mm, d98_d18 = 0 mm, d99_d19 = 0 mm, d100_d20 = 0 mm, d101_d1 = 0 mm, d102_d2 = 0 mm, d103_d3 = 0 mm, d104_d4 = 0 mm, d105_d5 = 0 mm, d106_d6 = 0 mm, d107_d7 = 0 mm, d108_d8 = 0 mm, d109_d9 = 0 mm, d110_d10 = 0 mm, d111_d0 = 0 mm
